# Autodesk Inventor assembly: field
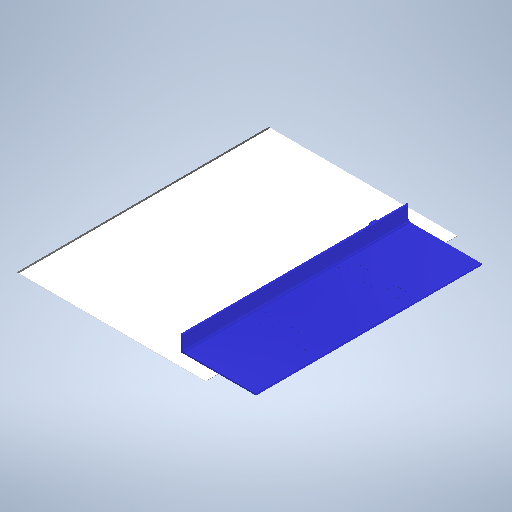
[picture p0: Inventor's stored thumbnail of the model, 512x512]
Saved by Autodesk Inventor 2025 (Build 290162000, 162)
## iProperties
Created: 2026-02-16
Part Number: field
Document SubType Name: Assembly
Designer: sooo1
Author: sooo1
## Documents named in this file (4)
- C:\Users\sooo1\Downloads\final-20260216T060151Z-1-001\final\field\field.iam
- C:\Users\sooo1\Downloads\final-20260216T060151Z-1-001\final\field\field_plate_SUS430.ipt
- C:\Users\sooo1\Downloads\final-20260216T060151Z-1-001\final\field\field_surface_paper.ipt
- C:\Users\sooo1\Downloads\final-20260216T060151Z-1-001\final\field\protectar.iam
## Components (3 placed, 3 different names)
1. field_plate_SUS430:1 — フラッシュ:1, フラッシュ:2, フラッシュ:3, メイト:1, メイト:2, フラッシュ:4, フラッシュ:5, フラッシュ:6
2. field_surface_paper:1 — メイト:1, メイト:2, フラッシュ:4, メイト:3
3. protectar:1 [sub-assembly] — メイト:3, フラッシュ:5, フラッシュ:6
## Relationships (9: Flush 6, Mate 3)
- フラッシュ:1 [Flush]: field_plate_SUS430:1
- フラッシュ:2 [Flush]: field_plate_SUS430:1
- フラッシュ:3 [Flush]: field_plate_SUS430:1
- メイト:1 [Mate]: field_plate_SUS430:1 ↔ field_surface_paper:1
- メイト:2 [Mate]: field_plate_SUS430:1 ↔ field_surface_paper:1
- フラッシュ:4 [Flush]: field_plate_SUS430:1 ↔ field_surface_paper:1
- メイト:3 [Mate]: field_surface_paper:1 ↔ protectar:1
- フラッシュ:5 [Flush]: field_plate_SUS430:1 ↔ protectar:1
- フラッシュ:6 [Flush] (60 mm): field_plate_SUS430:1 ↔ protectar:1
